# Autodesk Inventor assembly: camera_hausing
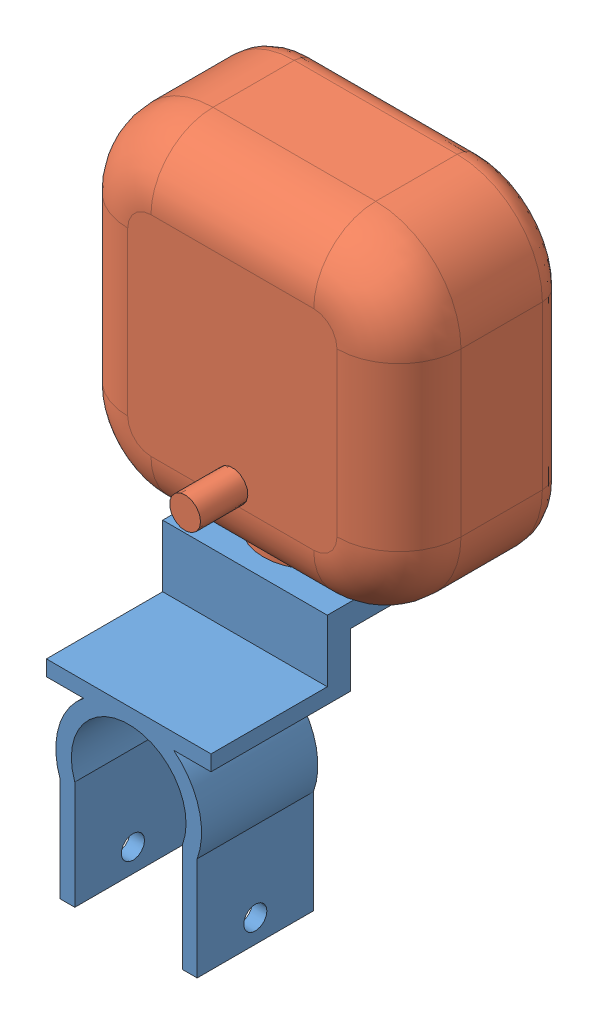
[picture p0: shaded view drawn from the part files that the assembly names]
Saved by Autodesk Inventor 2026.1 (Build 301233020, 233B)
## iProperties
Created: 2025-12-04
Part Number: camera_hausing
Document SubType Name: Assembly
Designer: jaewook
Author: jaewook
## Documents named in this file (3)
- C:\Users\kjh19\Documents\Inventor\project\turrte_projict_v2\camera_hausing.iam
- C:\Users\kjh19\Documents\Inventor\project\turrte_projict_v2\camera_base.ipt
- C:\Users\kjh19\Documents\Inventor\project\turrte_projict_v2\camera.ipt
## Components (2 placed, 2 different names)
1. camera_base:1 — 플러쉬:1, 플러쉬:2
2. camera:1 — 플러쉬:1, 플러쉬:2
## Relationships (2: Flush 2)
- 플러쉬:1 [Flush]: camera_base:1 ↔ camera:1
- 플러쉬:2 [Flush]: camera_base:1 ↔ camera:1
